# Autodesk Inventor assembly: leg5
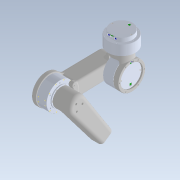
[picture p0: Inventor's stored thumbnail of the model, 180x180]
Saved by Autodesk Inventor 2020 (Build 240168000, 168)
## iProperties
Created: 2020-12-24
Part Number: leg5
Document SubType Name: Assembly
Designer: DELL
Author: DELL
## Documents named in this file (6)
- F:\SoftRobot2.0\Flexipod2.0\leg5_2020_12_24_11_46\leg5.iam
- F:\SoftRobot2.0\Flexipod2.0\RMD_X6_stator.ipt
- F:\SoftRobot2.0\Flexipod2.0\RMD_X6_rotor.ipt
- F:\SoftRobot2.0\Flexipod2.0\leg5_2020_12_24_11_46\shank_link.ipt
- F:\SoftRobot2.0\Flexipod2.0\leg5_2020_12_24_11_46\hip_link.ipt
- F:\SoftRobot2.0\Flexipod2.0\leg5_2020_12_24_11_46\shank_link_2.ipt
## Components (9 placed, 5 different names)
1. RMD_X6_stator:1 — Mate:1, Flush:1, Mate:7, Mate:8, Mate:9, Mate:10
2. RMD_X6_rotor:1 — Mate:1, Flush:1, Mate:11, Mate:12
3. RMD_X6_stator:2 — Mate:2, Flush:2, Mate:13, Mate:14, Mate:15, Mate:16, Mate:18, Angle:1
4. RMD_X6_rotor:2 — Mate:2, Flush:2, Mate:17, Mate:19
5. RMD_X6_stator:3 — Mate:4, Mate:20, Mate:22, Mate:23
6. RMD_X6_rotor:3 — Mate:5, Mate:6
7. shank_link:1 — Mate:4, Mate:5, Mate:6
8. hip_link:1 — Mate:10, Mate:11, Mate:12, Mate:13, Mate:14, Mate:15
9. shank_link_2:1 — Mate:16, Mate:17, Mate:18, Mate:19, Mate:20, Mate:22, Mate:23
## Relationships (26: Mate 22, Flush 3, Angle 1)
- Mate:1: RMD_X6_stator:1 ↔ RMD_X6_rotor:1
- Flush:1 (-3 mm): RMD_X6_stator:1 ↔ RMD_X6_rotor:1
- Mate:2: RMD_X6_stator:2 ↔ RMD_X6_rotor:2
- Flush:2 (-3 mm): RMD_X6_stator:2 ↔ RMD_X6_rotor:2
- [Mate]: RMD_X6_stator:3 ↔ RMD_X6_rotor:3
- [Flush] (-3 mm): RMD_X6_stator:3 ↔ RMD_X6_rotor:3
- Mate:4: RMD_X6_stator:3 ↔ shank_link:1
- Mate:5: RMD_X6_rotor:3 ↔ shank_link:1
- Mate:6: RMD_X6_rotor:3 ↔ shank_link:1
- Mate:7: RMD_X6_stator:1
- Mate:8: RMD_X6_stator:1
- Mate:9: RMD_X6_stator:1
- Mate:10: RMD_X6_stator:1 ↔ hip_link:1
- Mate:11: RMD_X6_rotor:1 ↔ hip_link:1
- Mate:12: RMD_X6_rotor:1 ↔ hip_link:1
- Mate:13: RMD_X6_stator:2 ↔ hip_link:1
- Mate:14: RMD_X6_stator:2 ↔ hip_link:1
- Mate:15: RMD_X6_stator:2 ↔ hip_link:1
- Mate:16: RMD_X6_stator:2 ↔ shank_link_2:1
- Mate:17: RMD_X6_rotor:2 ↔ shank_link_2:1
- Mate:18: RMD_X6_stator:2 ↔ shank_link_2:1
- Mate:19: RMD_X6_rotor:2 ↔ shank_link_2:1
- Mate:20: RMD_X6_stator:3 ↔ shank_link_2:1
- Mate:22: RMD_X6_stator:3 ↔ shank_link_2:1
- Angle:1 (0 deg): RMD_X6_stator:2
- Mate:23: RMD_X6_stator:3 ↔ shank_link_2:1
## Named parameters: d4_d2 = 0 mm, d5_d3 = -3 mm
